# Autodesk Inventor assembly: Pa1[2]
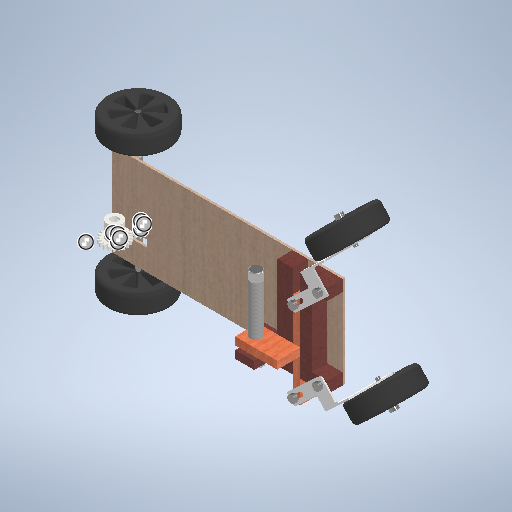
[picture p0: Inventor's stored thumbnail of the model, 512x512]
Saved by Autodesk Inventor 2025.2 (Build 292293000, 293)
## iProperties
Created: 2025-02-15
Part Number: Pa1[2]
Document SubType Name: Assembly
Designer: shiva
Author: shiva
## Documents named in this file (15)
- C:\Users\mpava\OneDrive - IIT Kanpur\TA212_group35\MPK's_work\Pa1[2].iam
- C:\Users\mpava\OneDrive - IIT Kanpur\TA212_group35\MPK's_work\base_01[1].ipt
- C:\Users\mpava\OneDrive - IIT Kanpur\TA212_group35\MPK's_work\front_U_shaped_frame[1].ipt
- C:\Users\mpava\OneDrive - IIT Kanpur\TA212_group35\MPK's_work\steering_connector[1].ipt
- C:\Users\mpava\OneDrive - IIT Kanpur\TA212_group35\MPK's_work\steering_helper_base[1].ipt
- C:\Users\mpava\OneDrive - IIT Kanpur\TA212_group35\MPK's_work\Bolt.ipt
- C:\Users\mpava\OneDrive - IIT Kanpur\TA212_group35\MPK's_work\tyreta212[1].ipt
- C:\Users\mpava\OneDrive - IIT Kanpur\TA212_group35\MPK's_work\Bolt 2.ipt
- C:\Users\mpava\OneDrive - IIT Kanpur\TA212_group35\MPK's_work\Rectangle_plate[1].ipt
- C:\Users\mpava\OneDrive - IIT Kanpur\TA212_group35\MPK's_work\Main Bolt.ipt
- C:\Users\mpava\OneDrive - IIT Kanpur\TA212_group35\MPK's_work\Main Shaft.ipt
- C:\Users\mpava\OneDrive - IIT Kanpur\TA212_group35\MPK's_work\Holder for Main_Shaft.ipt
- C:\Users\mpava\OneDrive - IIT Kanpur\TA212_group35\MPK's_work\Holder for Main_Shaft_MIR.ipt
- C:\Users\mpava\OneDrive - IIT Kanpur\TA212_group35\MPK's_work\Rectangle_plate[1]_MIR1.ipt
- C:\Users\mpava\OneDrive\Desktop\Spur Gears\Design Accelerator\Spur Gear11.ipt
## Components (22 placed, 14 different names)
1. base_01[1]:1 — Mate:2, Flush:3, Flush:4, Flush:5, Flush:6, Flush:8, Mate:48, Mate:49, Flush:14, Mate:61, Mate:65, Mate:66
2. front_U_shaped_frame[1]:1 — Flush:4, Flush:5, Mate:6, Mate:17, Mate:18, Mate:25, Mate:53, Mate:54, Mate:66
3. steering_connector[1]:1 — Mate:2, Mate:5, Mate:6, Mate:12, Mate:14
4. steering_helper_base[1]:1 — Flush:3, Mate:5, Mate:35, Mate:36, Mate:65
5. Bolt:1 — Mate:14, Mate:55, Tangent:2
6. Bolt:2 — Mate:12, Tangent:1, Mate:31
7. Bolt:3 — Mate:17, Mate:26, Mate:32
8. Bolt:4 — Mate:18, Mate:56
9. tyreta212[1]:1 — Mate:20, Mate:22, Mate:24, Rotation:6
10. tyreta212[1]:2 — Mate:19, Mate:21, Rotation:7, Mate:52
11. Bolt 2:1 — Mate:20, Mate:22, Mate:50
12. Bolt 2:2 — Mate:19, Mate:21, Mate:51
13. Rectangle_plate[1]:1 — Mate:24, Mate:25, Mate:26, Tangent:1, Mate:31, Mate:32, Rotation:1, Mate:50
14. Main Bolt:1 — Mate:35, Mate:36, Rotation:1
15. Main Shaft:1 — Mate:39, Mate:44, Mate:45, Mate:46, Flush:12, Flush:13, Rotation:4, Rotation:5, Rotation:6, Rotation:7, Mate:47, Mate:60
16. Holder for Main_Shaft:1 — Flush:6, Mate:39, Mate:46, Mate:48, Flush:14
17. Holder for Main_Shaft_MIR:1 — Flush:8, Mate:47, Mate:49
18. tyreta212[1]:3 — Mate:44, Flush:13, Rotation:4
19. tyreta212[1]:4 — Mate:45, Flush:12, Rotation:5
20. Rectangle_plate[1]_MIR1:1 — Mate:51, Mate:52, Mate:53, Mate:54, Mate:55, Mate:56, Tangent:2
21. Spur Gear1:1 — Mate:60, Mate:61, Mate:63, Mate:64
22. Spur Gear1:2 — Mate:63, Mate:64
## Relationships (53: Mate 38, Flush 8, RelateRotation 5, Tangent 2)
- Mate:2: base_01[1]:1 ↔ steering_connector[1]:1
- Flush:3: base_01[1]:1 ↔ steering_helper_base[1]:1
- Mate:5: steering_connector[1]:1 ↔ steering_helper_base[1]:1
- Flush:4: base_01[1]:1 ↔ front_U_shaped_frame[1]:1
- Flush:5: base_01[1]:1 ↔ front_U_shaped_frame[1]:1
- Mate:6: front_U_shaped_frame[1]:1 ↔ steering_connector[1]:1
- Mate:12: steering_connector[1]:1 ↔ Bolt:2
- Mate:14: steering_connector[1]:1 ↔ Bolt:1
- Mate:17: front_U_shaped_frame[1]:1 ↔ Bolt:3
- Mate:18: front_U_shaped_frame[1]:1 ↔ Bolt:4
- Mate:19: tyreta212[1]:2 ↔ Bolt 2:2
- Mate:20: tyreta212[1]:1 ↔ Bolt 2:1
- Mate:21: tyreta212[1]:2 ↔ Bolt 2:2
- Mate:22: tyreta212[1]:1 ↔ Bolt 2:1
- Mate:24: tyreta212[1]:1 ↔ Rectangle_plate[1]:1
- Mate:25: front_U_shaped_frame[1]:1 ↔ Rectangle_plate[1]:1
- Mate:26: Bolt:3 ↔ Rectangle_plate[1]:1
- Tangent:1: Bolt:2 ↔ Rectangle_plate[1]:1
- Mate:31: Bolt:2 ↔ Rectangle_plate[1]:1
- Mate:32: Bolt:3 ↔ Rectangle_plate[1]:1
- Mate:35: steering_helper_base[1]:1 ↔ Main Bolt:1
- Mate:36: steering_helper_base[1]:1 ↔ Main Bolt:1
- Rotation:1 [RelateRotation] (200 ul): Rectangle_plate[1]:1 ↔ Main Bolt:1
- Flush:6: base_01[1]:1 ↔ Holder for Main_Shaft:1
- Mate:39: Main Shaft:1 ↔ Holder for Main_Shaft:1
- Flush:8: base_01[1]:1 ↔ Holder for Main_Shaft_MIR:1
- Mate:44: Main Shaft:1 ↔ tyreta212[1]:3
- Mate:45: Main Shaft:1 ↔ tyreta212[1]:4
- Mate:46: Main Shaft:1 ↔ Holder for Main_Shaft:1
- Flush:12: Main Shaft:1 ↔ tyreta212[1]:4
- Flush:13: Main Shaft:1 ↔ tyreta212[1]:3
- Rotation:4 [RelateRotation] (1 ul): Main Shaft:1 ↔ tyreta212[1]:3
- Rotation:5 [RelateRotation] (1 ul): Main Shaft:1 ↔ tyreta212[1]:4
- Rotation:6 [RelateRotation] (1 ul): tyreta212[1]:1 ↔ Main Shaft:1
- Rotation:7 [RelateRotation] (1 ul): tyreta212[1]:2 ↔ Main Shaft:1
- Mate:47: Main Shaft:1 ↔ Holder for Main_Shaft_MIR:1
- Mate:48: base_01[1]:1 ↔ Holder for Main_Shaft:1
- Mate:49: base_01[1]:1 ↔ Holder for Main_Shaft_MIR:1
- Flush:14 (10 mm): base_01[1]:1 ↔ Holder for Main_Shaft:1
- Mate:50: Bolt 2:1 ↔ Rectangle_plate[1]:1
- Mate:51: Bolt 2:2 ↔ Rectangle_plate[1]_MIR1:1
- Mate:52: tyreta212[1]:2 ↔ Rectangle_plate[1]_MIR1:1
- Mate:53: front_U_shaped_frame[1]:1 ↔ Rectangle_plate[1]_MIR1:1
- Mate:54: front_U_shaped_frame[1]:1 ↔ Rectangle_plate[1]_MIR1:1
- Mate:55: Bolt:1 ↔ Rectangle_plate[1]_MIR1:1
- Mate:56: Bolt:4 ↔ Rectangle_plate[1]_MIR1:1
- Tangent:2: Bolt:1 ↔ Rectangle_plate[1]_MIR1:1
- Mate:60: Main Shaft:1 ↔ Spur Gear1:1
- Mate:61 (2 mm): base_01[1]:1 ↔ Spur Gear1:1
- Mate:63 (30 mm): Spur Gear1:1 ↔ Spur Gear1:2
- Mate:64: Spur Gear1:1 ↔ Spur Gear1:2
- Mate:65: base_01[1]:1 ↔ steering_helper_base[1]:1
- Mate:66: base_01[1]:1 ↔ front_U_shaped_frame[1]:1
